# Autodesk Inventor assembly: LED
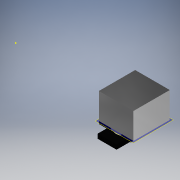
[picture p0: Inventor's stored thumbnail of the model, 180x180]
Saved by Autodesk Inventor 2016 (Build 200138000, 138)
## iProperties
Created: 2016-11-08
Part Number: LED
Material: Generisch
Document SubType Name: Assembly
Designer: Bene
Author: Bene
## Documents named in this file (5)
- C:\Users\Bene\Dropbox\Dokumente\OpticalDesign\Beamerscope\Inventor\Beamerscope_r4\LED.iam
- C:\Users\Bene\Dropbox\Dokumente\OpticalDesign\Beamerscope\Inventor\Beamerscope_r4\01_Coolingblock.ipt
- C:\Users\Bene\Dropbox\Dokumente\OpticalDesign\Beamerscope\Inventor\Beamerscope_r4\03_LED.ipt
- C:\Users\Bene\Dropbox\Dokumente\OpticalDesign\Beamerscope\Inventor\Beamerscope_r4\04_LED_Holder.ipt
- C:\Users\Bene\Dropbox\Dokumente\OpticalDesign\Beamerscope\Inventor\Beamerscope_r4\05_Collimator.ipt
## Components (4 placed, 4 different names)
1. 01_Coolingblock:1 — Fluchtend:3, Fluchtend:4, Fluchtend:5, Fluchtend:6
2. 03_LED:1 — Fluchtend:3, Fluchtend:4
3. 04_LED_Holder:1 — Fluchtend:5, Fluchtend:6, Fluchtend:7
4. 05_Collimator:1 — Fluchtend:7
## Relationships (5: Flush 5)
- Fluchtend:3 [Flush]: 01_Coolingblock:1 ↔ 03_LED:1
- Fluchtend:4 [Flush]: 01_Coolingblock:1 ↔ 03_LED:1
- Fluchtend:5 [Flush]: 01_Coolingblock:1 ↔ 04_LED_Holder:1
- Fluchtend:6 [Flush]: 01_Coolingblock:1 ↔ 04_LED_Holder:1
- Fluchtend:7 [Flush]: 04_LED_Holder:1 ↔ 05_Collimator:1
